# Autodesk Inventor assembly: Gear Box Assembly 2
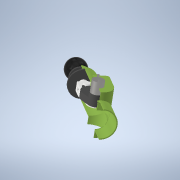
[picture p0: Inventor's stored thumbnail of the model, 180x180]
Saved by Autodesk Inventor 2022 (Build 260153000, 153)
## iProperties
Created: 2023-01-26
Part Number: Gear Box Assembly 2
Document SubType Name: Assembly
Designer: ASUS
Author: ASUS
## Documents named in this file (13)
- C:\Users\ASUS\Documents\Design Portfolio\Massage Gun\Internals\Gear Box Assembly 2.iam
- C:\Users\ASUS\Documents\Design Portfolio\Massage Gun\Internals\Gear Box Shell.ipt
- C:\Users\ASUS\Documents\Design Portfolio\Air Pump\Internal parts\Motor.ipt
- C:\Users\ASUS\Documents\Design Portfolio\Massage Gun\Internals\Untitled.iam
- C:\Users\ASUS\Documents\Design Portfolio\Massage Gun\Internals\Bearing.ipt
- C:\Users\ASUS\Documents\Design Portfolio\Massage Gun\Internals\Drive Gear.iam
- C:\Users\ASUS\Documents\Design Portfolio\Massage Gun\Internals\Push Rod v2.ipt
- C:\Users\ASUS\Documents\Design Portfolio\Massage Gun\Internals\Bearing rod.ipt
- C:\Users\ASUS\Documents\Design Portfolio\Massage Gun\Internals\Push Rod Holder.ipt
- C:\Users\ASUS\Documents\Design Portfolio\Massage Gun\Internals\Shell V2.ipt
- C:\Users\ASUS\Documents\Design Portfolio\Massage Gun\Internals\Piston.ipt
- C:\Users\ASUS\Documents\Design Portfolio\Massage Gun\Internals\Small Push Rod Holder.ipt
- C:\Users\ASUS\Documents\Design Portfolio\Massage Gun\Internals\Ball.ipt
## Components (16 placed, 12 different names)
1. Motor:1 — Rotational:2, Mate:14
2. Drive Gear:1 [sub-assembly] — Rotational:2
3. Push Rod v2:1 — Mate:12, Rotational:13, Rotational:14, Mate:17, Mate:18, Mate:19
4. Bearing:3 — Rotational:13
5. Bearing rod:1 — Rigid:3
6. Push Rod Holder:1 — Mate:9, Mate:10
7. Shell V2:1 — Mate:9, Mate:10, Mate:12, Mate:13, Flush:3, Mate:15, Mate:16
8. Bearing:5 — Rotational:14, Rigid:3, Rotational:18
9. Gear Box Shell:1 — Mate:13, Mate:14, Flush:3, Mate:15, Rotational:19
10. Bearing:6 — Flush:2, Rotational:15, Rotational:19
11. Untitled:1 [sub-assembly] — Flush:2, Rotational:15, Rotational:17
12. Piston:1 — Rigid:2, Rotational:16
13. Bearing:7 — Rigid:2, Rotational:18
14. Bearing:8 — Rotational:16, Rotational:17
15. Small Push Rod Holder:1 — Mate:16, Mate:17
16. Ball:1 — Mate:18, Mate:19
## Relationships (22: Mate 10, RevoluteJoint 8, Flush 2, WeldJoint 2)
- Rotational:2 [RevoluteJoint]: Motor:1 ↔ Drive Gear:1
- Mate:9: Push Rod Holder:1 ↔ Shell V2:1
- Mate:10: Push Rod Holder:1 ↔ Shell V2:1
- Mate:12: Push Rod v2:1 ↔ Shell V2:1
- Rotational:13 [RevoluteJoint]: Push Rod v2:1 ↔ Bearing:3
- Rotational:14 [RevoluteJoint]: Push Rod v2:1 ↔ Bearing:5
- Flush:2: Bearing:6 ↔ Untitled:1
- Rotational:15 [RevoluteJoint]: Bearing:6 ↔ Untitled:1
- Rigid:2 [WeldJoint]: Piston:1 ↔ Bearing:7
- Rotational:16 [RevoluteJoint]: Piston:1 ↔ Bearing:8
- Rotational:17 [RevoluteJoint]: Untitled:1 ↔ Bearing:8
- Rigid:3 [WeldJoint]: Bearing rod:1 ↔ Bearing:5
- Rotational:18 [RevoluteJoint]: Bearing:5 ↔ Bearing:7
- Mate:13: Shell V2:1 ↔ Gear Box Shell:1
- Mate:14: Motor:1 ↔ Gear Box Shell:1
- Flush:3: Shell V2:1 ↔ Gear Box Shell:1
- Mate:15: Shell V2:1 ↔ Gear Box Shell:1
- Rotational:19 [RevoluteJoint]: Gear Box Shell:1 ↔ Bearing:6
- Mate:16: Shell V2:1 ↔ Small Push Rod Holder:1
- Mate:17: Push Rod v2:1 ↔ Small Push Rod Holder:1
- Mate:18: Push Rod v2:1 ↔ Ball:1
- Mate:19: Push Rod v2:1 ↔ Ball:1
